# Autodesk Inventor assembly: MOGO Funnel
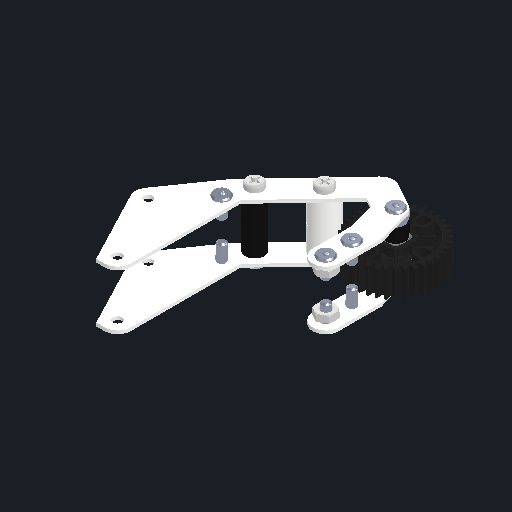
[picture p0: Inventor's stored thumbnail of the model, 512x512]
Saved by Autodesk Inventor 2025 (Build 290162000, 162)
## iProperties
Created: 2024-12-17
Part Number: MOGO Funnel
Document SubType Name: Assembly
Designer: avere
Author: Averey Ku
## Documents named in this file (19)
- D:\VEX\High Stakes\CAD\V4\Chassis\Drivebay Left\MOGO Funnel.iam
- D:\VEX\High Stakes\CAD\V4\Chassis\Drivebay Right\Ring Funnel.ipt
- D:\VEX\High Stakes\CAD\ROBOPROS-CAD-Inventor\Motion\Spacers\Spacer Nylon .375 OD\NSpacer .375 OD x .500.ipt
- D:\VEX\High Stakes\CAD\ROBOPROS-CAD-Inventor\Motion\Spacers\Spacer Nylon .500 OD\NSpacer White .500 OD x .500.ipt
- D:\VEX\High Stakes\CAD\V4\Chassis\Drivebay Right\HS 36T Gear, No Insert.iam
- D:\VEX\High Stakes\CAD\V4\Chassis\Drivebay Right\NScrew Pan Head Threaded 1.250.ipt
- D:\VEX\High Stakes\CAD\ROBOPROS-CAD-Inventor\Structure\Hardware\Screw Steel - Star\SScrew Star Smooth 1.250.ipt
- D:\VEX\High Stakes\CAD\V4\Chassis\Drivebay Right\Nut Nylon Thread-Forming.ipt
- D:\VEX\High Stakes\CAD\ROBOPROS-CAD-Inventor\Structure\Hardware\Screw Shoulder Robosource\SScrew Shoulder Smooth .375 x .12.ipt
- D:\VEX\High Stakes\CAD\ROBOPROS-CAD-Inventor\Motion\Spacers\Washer Steel\SWasher .375 OD x .062500.ipt
- D:\VEX\High Stakes\CAD\ROBOPROS-CAD-Inventor\Motion\Spacers\Washer Steel\SWasher .375 OD x .031250.ipt
- D:\VEX\High Stakes\CAD\V4\Chassis\Drivebay Right\Nut Keps.ipt
- D:\VEX\High Stakes\CAD\ROBOPROS-CAD-Inventor\Motion\Spacers\Spacer Nylon .375 OD\NSpacer .375 OD x .250.ipt
- D:\VEX\High Stakes\CAD\ROBOPROS-CAD-Inventor\Motion\Spacers\Spacer Nylon .375 OD.ipt
- D:\VEX\High Stakes\CAD\ROBOPROS-CAD-Inventor\Motion\Spacers\Spacer Nylon .500 OD.ipt
- D:\VEX\High Stakes\CAD\ROBOPROS-CAD-Inventor\Structure\Hardware\Screw Steel - Star.ipt
- D:\VEX\High Stakes\CAD\ROBOPROS-CAD-Inventor\Structure\Hardware\Screw Shoulder Robosource.ipt
- D:\VEX\High Stakes\CAD\ROBOPROS-CAD-Inventor\Motion\Spacers\Washer Steel.ipt
- D:\VEX\High Stakes\CAD\V4\Chassis\Drivebay Left\Custom Parts\MOGO Funnel.ipt
## Components (28 placed, 13 different names)
1. Ring Funnel:1 — Mate:1, Insert:1, Insert:3, Insert:5, Insert:9, Insert:11, Insert:12, Insert:19, Insert:17, Insert:18, Insert:23, Insert:27, Insert:30, Mate:2
2. Ring Funnel:2 — Mate:1, Insert:1, Insert:6, Insert:13, Insert:15, Insert:16, Insert:21, Insert:20, Insert:22, Insert:24, Insert:26, Insert:31, Mate:3
3. NSpacer .375 OD x .500:1 — Insert:2
4. NSpacer .375 OD x .500:2 — Insert:3, Insert:2
5. NSpacer White .500 OD x .500:1 — Insert:4
6. NSpacer White .500 OD x .500:2 — Insert:5, Insert:4
7. HS 36T Gear, No Insert:1 [sub-assembly] — Insert:6
8. NScrew Pan Head Threaded 1.250:2 — Insert:9
9. SScrew Star Smooth 1.250:1 — Insert:11
10. NScrew Pan Head Threaded 1.250:3 — Insert:12
11. Nut Nylon Thread-Forming:1 — Insert:13
12. Nut Nylon Thread-Forming:3 — Insert:15
13. Nut Nylon Thread-Forming:4 — Insert:16
14. SScrew Shoulder Smooth .375 x .12:1 — Insert:19
15. SScrew Shoulder Smooth .375 x .12:2 — Insert:17
16. SScrew Shoulder Smooth .375 x .12:3 — Insert:18
17. SScrew Shoulder Smooth .375 x .12:4 — Insert:21
18. SScrew Shoulder Smooth .375 x .12:5 — Insert:20
19. SScrew Shoulder Smooth .375 x .12:6 — Insert:22
20. Nut Nylon Thread-Forming:5 — Insert:23
21. Nut Nylon Thread-Forming:6 — Insert:24
22. SWasher .375 OD x .062500:1 — Insert:26, Insert:25
23. SWasher .375 OD x .031250:2 — Insert:25
24. Nut Keps:1 — Insert:27, Insert:29
25. SWasher .375 OD x .062500:3 — Insert:28
26. NSpacer .375 OD x .250:3 — Insert:29, Insert:28
27. MOGO Funnel:1 — Insert:30, Mate:2
28. MOGO Funnel:2 — Insert:31, Mate:3
## Relationships (30: Insert 27, Mate 3)
- Mate:1: Ring Funnel:1 ↔ Ring Funnel:2
- Insert:1 (25.4 mm): Ring Funnel:1 ↔ Ring Funnel:2
- Insert:3: Ring Funnel:1 ↔ NSpacer .375 OD x .500:2
- Insert:2: NSpacer .375 OD x .500:1 ↔ NSpacer .375 OD x .500:2
- Insert:5: Ring Funnel:1 ↔ NSpacer White .500 OD x .500:2
- Insert:4: NSpacer White .500 OD x .500:1 ↔ NSpacer White .500 OD x .500:2
- Insert:6 (2.3813 mm): Ring Funnel:2 ↔ HS 36T Gear, No Insert:1
- Insert:9: Ring Funnel:1 ↔ NScrew Pan Head Threaded 1.250:2
- Insert:11: Ring Funnel:1 ↔ SScrew Star Smooth 1.250:1
- Insert:12: Ring Funnel:1 ↔ NScrew Pan Head Threaded 1.250:3
- Insert:13: Ring Funnel:2 ↔ Nut Nylon Thread-Forming:1
- Insert:15: Ring Funnel:2 ↔ Nut Nylon Thread-Forming:3
- Insert:16: Ring Funnel:2 ↔ Nut Nylon Thread-Forming:4
- Insert:19: Ring Funnel:1 ↔ SScrew Shoulder Smooth .375 x .12:1
- Insert:17: Ring Funnel:1 ↔ SScrew Shoulder Smooth .375 x .12:2
- Insert:18: Ring Funnel:1 ↔ SScrew Shoulder Smooth .375 x .12:3
- Insert:21: Ring Funnel:2 ↔ SScrew Shoulder Smooth .375 x .12:4
- Insert:20: Ring Funnel:2 ↔ SScrew Shoulder Smooth .375 x .12:5
- Insert:22: Ring Funnel:2 ↔ SScrew Shoulder Smooth .375 x .12:6
- Insert:23 (1.5875 mm): Ring Funnel:1 ↔ Nut Nylon Thread-Forming:5
- Insert:24 (1.5875 mm): Ring Funnel:2 ↔ Nut Nylon Thread-Forming:6
- Insert:26: Ring Funnel:2 ↔ SWasher .375 OD x .062500:1
- Insert:25: SWasher .375 OD x .062500:1 ↔ SWasher .375 OD x .031250:2
- Insert:27: Ring Funnel:1 ↔ Nut Keps:1
- Insert:29: Nut Keps:1 ↔ NSpacer .375 OD x .250:3
- Insert:28: SWasher .375 OD x .062500:3 ↔ NSpacer .375 OD x .250:3
- Insert:30: Ring Funnel:1 ↔ MOGO Funnel:1
- Mate:2: Ring Funnel:1 ↔ MOGO Funnel:1
- Insert:31: Ring Funnel:2 ↔ MOGO Funnel:2
- Mate:3: Ring Funnel:2 ↔ MOGO Funnel:2
